# Autodesk Inventor assembly: ZespolSilnika
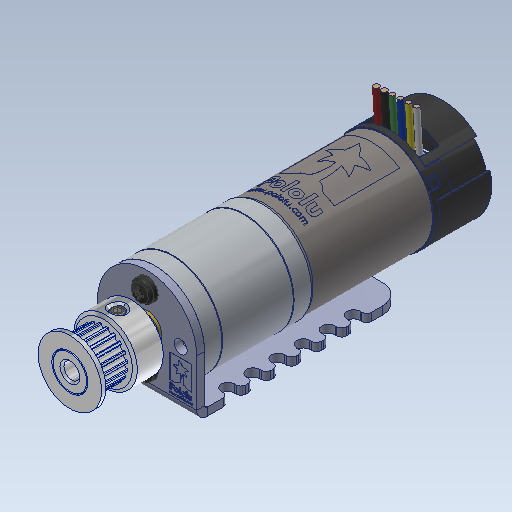
[picture p0: Inventor's stored thumbnail of the model, 512x512]
Saved by Autodesk Inventor 2020 (Build 240168000, 168)
## iProperties
Created: 2020-05-23
Part Number: ZespolSilnika
Document SubType Name: Assembly
Designer: estee
Author: estee
## Documents named in this file (6)
- C:\Users\Hesekiel\Desktop\MUM\Mechanika\Moduł obrotu RET Estera\prawieKoncowka\ModulSilnika.iam
- C:\Users\Hesekiel\Desktop\MUM\Mechanika\Moduł obrotu RET Estera\prawieKoncowka\kolooooo2.ipt
- C:\Users\Hesekiel\Desktop\MUM\Mechanika\Moduł obrotu RET Estera\prawieKoncowka\silnik25d-metal-gearmotor-378-499-encoder.ipt
- C:\Users\Hesekiel\Desktop\MUM\Mechanika\Moduł obrotu RET Estera\prawieKoncowka\trzymakpololu-25d-mm-metal-gearmotor-bracket.ipt
- C:\Users\Hesekiel\Desktop\MUM\Mechanika\Moduł obrotu RET Estera\prawieKoncowka\DIN EN ISO 7045 - M3 x 8 - 4.8 - Z.ipt
- C:\Users\Hesekiel\Desktop\MUM\Mechanika\Moduł obrotu RET Estera\prawieKoncowka\ISO 4029 - M3 x 6 - ISO.ipt
## Components (7 placed, 5 different names)
1. kolooooo2:1 — Mate:7, Mate:8, Mate:9, Mate:10
2. silnik25d-metal-gearmotor-378-499-encoder:1 — Mate:1, Mate:2, Mate:7, Tangent:1, Flush:1
3. trzymakpololu-25d-mm-metal-gearmotor-bracket:1 — Mate:1, Mate:2, Mate:3, Mate:4, Mate:5, Mate:6, Mate:8
4. DIN EN ISO 7045 Z M3 x 8 - 4.8 - Z:1 — Mate:3, Mate:6
5. DIN EN ISO 7045 Z M3 x 8 - 4.8 - Z:2 — Mate:4, Mate:5
6. ISO 4029 M3 x 6:1 — Mate:9, Flush:1
7. ISO 4029 M3 x 6:2 — Mate:10, Tangent:1
## Relationships (12: Mate 10, Tangent 1, Flush 1)
- Mate:1: silnik25d-metal-gearmotor-378-499-encoder:1 ↔ trzymakpololu-25d-mm-metal-gearmotor-bracket:1
- Mate:2: silnik25d-metal-gearmotor-378-499-encoder:1 ↔ trzymakpololu-25d-mm-metal-gearmotor-bracket:1
- Mate:3: trzymakpololu-25d-mm-metal-gearmotor-bracket:1 ↔ DIN EN ISO 7045 Z M3 x 8 - 4.8 - Z:1
- Mate:4: trzymakpololu-25d-mm-metal-gearmotor-bracket:1 ↔ DIN EN ISO 7045 Z M3 x 8 - 4.8 - Z:2
- Mate:5: trzymakpololu-25d-mm-metal-gearmotor-bracket:1 ↔ DIN EN ISO 7045 Z M3 x 8 - 4.8 - Z:2
- Mate:6: trzymakpololu-25d-mm-metal-gearmotor-bracket:1 ↔ DIN EN ISO 7045 Z M3 x 8 - 4.8 - Z:1
- Mate:7: kolooooo2:1 ↔ silnik25d-metal-gearmotor-378-499-encoder:1
- Mate:8 (3.5 mm): kolooooo2:1 ↔ trzymakpololu-25d-mm-metal-gearmotor-bracket:1
- Mate:9: kolooooo2:1 ↔ ISO 4029 M3 x 6:1
- Mate:10: kolooooo2:1 ↔ ISO 4029 M3 x 6:2
- Tangent:1 (-10 mm): silnik25d-metal-gearmotor-378-499-encoder:1 ↔ ISO 4029 M3 x 6:2
- Flush:1 (-6 mm): silnik25d-metal-gearmotor-378-499-encoder:1 ↔ ISO 4029 M3 x 6:1
